# Autodesk Inventor assembly: A2017_T4_04
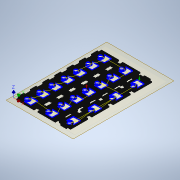
[picture p0: Inventor's stored thumbnail of the model, 180x180]
Saved by Autodesk Inventor 2022 (Build 260153000, 153)
## iProperties
Created: 2022-09-28
Part Number: A2017_T4_04
Document SubType Name: Assembly
Designer: Masato
Author: Masato
## Documents named in this file (3)
- C:\Users\6343y\ドキュメント\Inventor\SUSTAINA-OP\Cam\A2017_T4\A2017_T4_04.iam
- C:\Users\6343y\ドキュメント\Inventor\SUSTAINA-OP\Cam\DisposableBoard.ipt
- C:\Users\6343y\ドキュメント\Inventor\SUSTAINA-OP\UpperBody\Trunk\Trunk_servo_bottom_frame.ipt
## Components (19 placed, 2 different names)
1. DisposableBoard:1 — フラッシュ:1, フラッシュ:2, フラッシュ:3, フラッシュ:4, フラッシュ:7, フラッシュ:8, フラッシュ:9
2. Trunk_servo_bottom_frame:1 — メイト:3, フラッシュ:7, フラッシュ:8
3. Trunk_servo_bottom_frame:14 — メイト:5
4. Trunk_servo_bottom_frame:15
5. Trunk_servo_bottom_frame:16
6. Trunk_servo_bottom_frame:17
7. Trunk_servo_bottom_frame:18
8. Trunk_servo_bottom_frame:19
9. Trunk_servo_bottom_frame:20
10. Trunk_servo_bottom_frame:21
11. Trunk_servo_bottom_frame:22
12. Trunk_servo_bottom_frame:23
13. Trunk_servo_bottom_frame:24
14. Trunk_servo_bottom_frame:25
15. Trunk_servo_bottom_frame:26
16. Trunk_servo_bottom_frame:27 — メイト:4, メイト:5, フラッシュ:9
17. Trunk_servo_bottom_frame:28
18. Trunk_servo_bottom_frame:29
19. Trunk_servo_bottom_frame:30
## Component patterns: (14 elements, first: Trunk_servo_bottom_frame:1), (4 elements, first: Trunk_servo_bottom_frame:27)
## Relationships (10: Flush 7, Mate 3)
- フラッシュ:1 [Flush]: DisposableBoard:1
- フラッシュ:2 [Flush]: DisposableBoard:1
- フラッシュ:3 [Flush]: DisposableBoard:1
- フラッシュ:4 [Flush]: DisposableBoard:1
- メイト:3 [Mate]: Trunk_servo_bottom_frame:1
- フラッシュ:7 [Flush] (2.1 mm): DisposableBoard:1 ↔ Trunk_servo_bottom_frame:1
- フラッシュ:8 [Flush] (2.1 mm): DisposableBoard:1 ↔ Trunk_servo_bottom_frame:1
- メイト:4 [Mate]: Trunk_servo_bottom_frame:27
- メイト:5 [Mate] (2.1 mm): Trunk_servo_bottom_frame:14 ↔ Trunk_servo_bottom_frame:27
- フラッシュ:9 [Flush] (2.1 mm): DisposableBoard:1 ↔ Trunk_servo_bottom_frame:27
